# Autodesk Inventor assembly: roll_support_left_v1
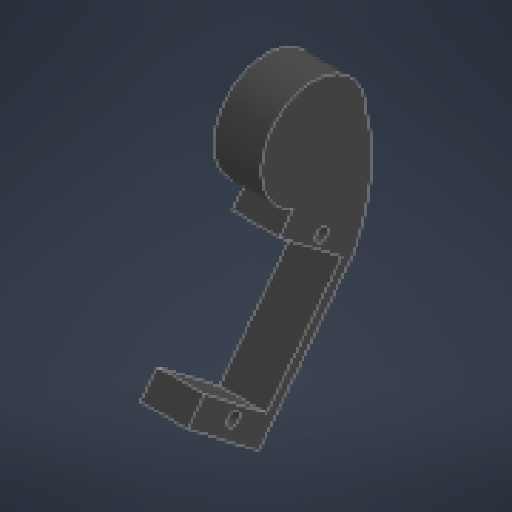
[picture p0: Inventor's stored thumbnail of the model, 512x512]
Saved by Autodesk Inventor 2026.1 (Build 301233020, 233B)
## iProperties
Created: 2025-11-28
Part Number: roll_support_left_v1
Document SubType Name: Assembly
Designer: jaewook
Author: jaewook
## Documents named in this file (3)
- C:\Users\kjh19\Documents\Inventor\project\turrte_projict_v2\roll_support_left_v1.iam
- C:\Users\kjh19\Documents\Inventor\project\turrte_projict_v2\support.ipt
- C:\Users\kjh19\Documents\Inventor\project\turrte_projict_v2\base_front.ipt
## Components (2 placed, 2 different names)
1. support:2 — 메이트:1
2. base_front:1 — 메이트:1
## Relationships (1: Mate 1)
- 메이트:1 [Mate]: support:2 ↔ base_front:1
